# Autodesk Inventor assembly: UpperArm_without_bumper
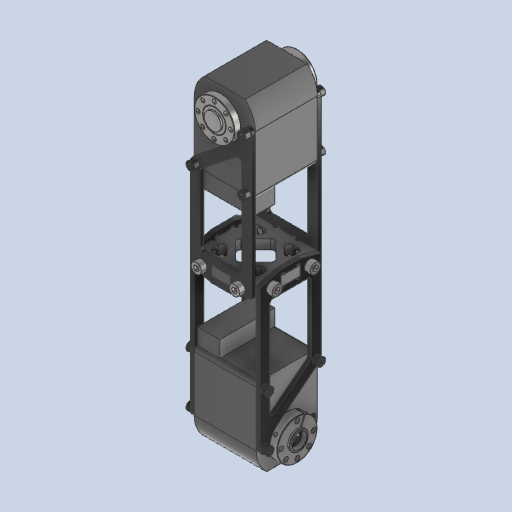
[picture p0: Inventor's stored thumbnail of the model, 512x512]
Saved by Autodesk Inventor 2022.5 (Build 265521000, 521)
## iProperties
Created: 2021-09-11
Part Number: UpperArm_without_bumper
Document SubType Name: Assembly
Designer: Masato
Mass: 132.402 g
Surface Area: 432.665 cm^2
Volume: 110.152 cm^3
Density: 1.20199 g/cm^3
Author: Masato
## Documents named in this file (7)
- C:\Users\Masato\Documents\Inventor\SUSTAINA-OP\ModelingFiles\UpperBody\Arm\UpperArm_without_bumper.iam
- C:\Users\Masato\Documents\Inventor\SUSTAINA-OP\ModelingFiles\UpperBody\Arm\UpperArm_side_frame.ipt
- C:\Users\Masato\Documents\Inventor\SUSTAINA-OP\ModelingFiles\COTS\Screw\FC-2615EB.ipt
- C:\Users\Masato\Documents\Inventor\SUSTAINA-OP\ModelingFiles\COTS\Screw\FC-2620EB.ipt
- C:\Users\Masato\Documents\Inventor\SUSTAINA-OP\ModelingFiles\COTS\Screw\UC-0306.ipt
- C:\Users\Masato\Documents\Inventor\SUSTAINA-OP\ModelingFiles\COTS\KONDO\B3M-SC-1040-A_with_ClampHorn_AND_FreeHorn.iam
- C:\Users\Masato\Documents\Inventor\SUSTAINA-OP\ModelingFiles\UpperBody\Arm\UpperArm_diagonal.iam
## Components (27 placed, 6 different names)
1. UpperArm_diagonal:1 [sub-assembly] — Insert:86, Insert:87, Insert:88, Insert:89, Insert:90, Insert:91, Insert:92, Insert:93
2. UpperArm_side_frame:1 — 挿入:32, 挿入:33, 挿入:34, 挿入:74, 挿入:75, 挿入:80, 挿入:84, 挿入:85, Insert:88, Insert:89
3. UpperArm_side_frame:2 — 挿入:11, 挿入:12, 挿入:38, 挿入:39, 挿入:40, 挿入:81, 挿入:82, 挿入:83, Insert:92, Insert:93
4. UpperArm_side_frame:3 — 挿入:14, 挿入:13, 挿入:35, 挿入:36, 挿入:37, 挿入:77, 挿入:78, 挿入:79, Insert:86, Insert:87
5. UpperArm_side_frame:4 — 挿入:15, 挿入:16, 挿入:29, 挿入:30, 挿入:31, 挿入:72, 挿入:73, 挿入:76, Insert:90, Insert:91
6. B3M-SC-1040-A_with_ClampHorn_AND_FreeHorn:1 [sub-assembly] — 挿入:72, 挿入:73, 挿入:76, 挿入:77, 挿入:78, 挿入:79
7. B3M-SC-1040-A_with_ClampHorn_AND_FreeHorn:2 [sub-assembly] — 挿入:74, 挿入:75, 挿入:80, 挿入:81, 挿入:82, 挿入:83
8. FC-2615EB:1 — 挿入:29
9. FC-2615EB:2 — 挿入:30
10. FC-2620EB:3 — 挿入:37
11. FC-2620EB:4 — 挿入:39
12. FC-2620EB:5 — 挿入:38
13. FC-2620EB:6 — 挿入:40
14. FC-2620EB:1 — 挿入:35
15. FC-2620EB:2 — 挿入:36
16. FC-2615EB:3 — 挿入:31
17. FC-2615EB:4 — 挿入:32
18. FC-2615EB:5 — 挿入:33
19. FC-2615EB:6 — 挿入:34
20. UC-0306:1 — 挿入:84
21. UC-0306:2 — 挿入:85
22. UC-0306:3 — 挿入:11
23. UC-0306:4 — 挿入:12
24. UC-0306:5 — 挿入:13
25. UC-0306:6 — 挿入:14
26. UC-0306:7 — 挿入:15
27. UC-0306:8 — 挿入:16
## Relationships (40: Insert 40)
- 挿入:11 [Insert]: UpperArm_side_frame:2 ↔ UC-0306:3
- 挿入:12 [Insert]: UpperArm_side_frame:2 ↔ UC-0306:4
- 挿入:13 [Insert]: UpperArm_side_frame:3 ↔ UC-0306:5
- 挿入:14 [Insert]: UpperArm_side_frame:3 ↔ UC-0306:6
- 挿入:15 [Insert]: UpperArm_side_frame:4 ↔ UC-0306:7
- 挿入:16 [Insert]: UpperArm_side_frame:4 ↔ UC-0306:8
- 挿入:29 [Insert]: UpperArm_side_frame:4 ↔ FC-2615EB:1
- 挿入:30 [Insert]: UpperArm_side_frame:4 ↔ FC-2615EB:2
- 挿入:31 [Insert]: UpperArm_side_frame:4 ↔ FC-2615EB:3
- 挿入:32 [Insert]: UpperArm_side_frame:1 ↔ FC-2615EB:4
- 挿入:33 [Insert]: UpperArm_side_frame:1 ↔ FC-2615EB:5
- 挿入:35 [Insert]: UpperArm_side_frame:3 ↔ FC-2620EB:1
- 挿入:34 [Insert]: UpperArm_side_frame:1 ↔ FC-2615EB:6
- 挿入:36 [Insert]: UpperArm_side_frame:3 ↔ FC-2620EB:2
- 挿入:37 [Insert]: UpperArm_side_frame:3 ↔ FC-2620EB:3
- 挿入:38 [Insert]: UpperArm_side_frame:2 ↔ FC-2620EB:5
- 挿入:39 [Insert]: UpperArm_side_frame:2 ↔ FC-2620EB:4
- 挿入:40 [Insert]: UpperArm_side_frame:2 ↔ FC-2620EB:6
- 挿入:72 [Insert]: UpperArm_side_frame:4 ↔ B3M-SC-1040-A_with_ClampHorn_AND_FreeHorn:1
- 挿入:73 [Insert]: UpperArm_side_frame:4 ↔ B3M-SC-1040-A_with_ClampHorn_AND_FreeHorn:1
- 挿入:74 [Insert]: UpperArm_side_frame:1 ↔ B3M-SC-1040-A_with_ClampHorn_AND_FreeHorn:2
- 挿入:75 [Insert]: UpperArm_side_frame:1 ↔ B3M-SC-1040-A_with_ClampHorn_AND_FreeHorn:2
- 挿入:76 [Insert]: UpperArm_side_frame:4 ↔ B3M-SC-1040-A_with_ClampHorn_AND_FreeHorn:1
- 挿入:77 [Insert]: UpperArm_side_frame:3 ↔ B3M-SC-1040-A_with_ClampHorn_AND_FreeHorn:1
- 挿入:78 [Insert]: UpperArm_side_frame:3 ↔ B3M-SC-1040-A_with_ClampHorn_AND_FreeHorn:1
- 挿入:79 [Insert]: UpperArm_side_frame:3 ↔ B3M-SC-1040-A_with_ClampHorn_AND_FreeHorn:1
- 挿入:80 [Insert]: UpperArm_side_frame:1 ↔ B3M-SC-1040-A_with_ClampHorn_AND_FreeHorn:2
- 挿入:81 [Insert]: UpperArm_side_frame:2 ↔ B3M-SC-1040-A_with_ClampHorn_AND_FreeHorn:2
- 挿入:82 [Insert]: UpperArm_side_frame:2 ↔ B3M-SC-1040-A_with_ClampHorn_AND_FreeHorn:2
- 挿入:83 [Insert]: UpperArm_side_frame:2 ↔ B3M-SC-1040-A_with_ClampHorn_AND_FreeHorn:2
- 挿入:84 [Insert]: UpperArm_side_frame:1 ↔ UC-0306:1
- 挿入:85 [Insert]: UpperArm_side_frame:1 ↔ UC-0306:2
- Insert:86: UpperArm_diagonal:1 ↔ UpperArm_side_frame:3
- Insert:87: UpperArm_diagonal:1 ↔ UpperArm_side_frame:3
- Insert:88: UpperArm_diagonal:1 ↔ UpperArm_side_frame:1
- Insert:89: UpperArm_diagonal:1 ↔ UpperArm_side_frame:1
- Insert:90: UpperArm_diagonal:1 ↔ UpperArm_side_frame:4
- Insert:91: UpperArm_diagonal:1 ↔ UpperArm_side_frame:4
- Insert:92: UpperArm_diagonal:1 ↔ UpperArm_side_frame:2
- Insert:93: UpperArm_diagonal:1 ↔ UpperArm_side_frame:2
